# Autodesk Inventor assembly: fourbarintakebearing
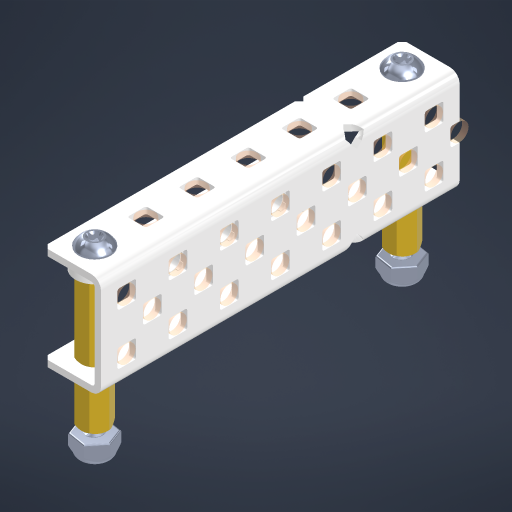
[picture p0: Inventor's stored thumbnail of the model, 512x512]
Saved by Autodesk Inventor 2023 (Build 270158000, 158)
## iProperties
Created: 2023-08-08
Part Number: fourbarintakebearing
Document SubType Name: Assembly
Designer: srbel
Author: srbel
## Documents named in this file (11)
- C:\CAD\OverUnderCAD\Drive\fourbarintakebearing.iam
- C:\CAD\OverUnderCAD\VEX-CAD-Inventor-1.4.0\Structure\C Channel\Aluminum 1x2x1\Alu C 1x2x1x7.ipt
- C:\CAD\OverUnderCAD\VEX-CAD-Inventor-1.4.0\Structure\Standoff\Standoff .50.ipt
- C:\CAD\OverUnderCAD\VEX-CAD-Inventor-1.4.0\Structure\Standoff.ipt
- C:\CAD\OverUnderCAD\VEX-CAD-Inventor-1.4.0\Motion\Spacers\Spacer Nylon .313 OD\NSpacer .313 OD x .125.ipt
- C:\CAD\OverUnderCAD\VEX-CAD-Inventor-1.4.0\Motion\Spacers\Spacer Nylon .313 OD.ipt
- C:\CAD\OverUnderCAD\VEX-CAD-Inventor-1.4.0\Structure\Standoff\Standoff .75.ipt
- C:\CAD\OverUnderCAD\VEX-CAD-Inventor-1.4.0\Motion\Shaft LS\Bearing Flat.ipt
- C:\CAD\OverUnderCAD\VEX-CAD-Inventor-1.4.0\Structure\Hardware\Screw Steel - Star.ipt
- C:\CAD\OverUnderCAD\VEX-CAD-Inventor-1.4.0\Structure\Hardware\Screw Steel - Star\SScrew Star Threaded 1.750.ipt
- C:\CAD\OverUnderCAD\VEX-CAD-Inventor-1.4.0\Structure\Hardware\Nut Thin Nylock.ipt
## Components (12 placed, 7 different names)
1. Alu C 1x2x1x7:1 — Insert:9, Insert:12
2. Standoff .50:1 — Insert:10
3. Standoff .50:2 — Insert:11
4. NSpacer .313 OD x .125:1
5. Standoff .75:3
6. NSpacer .313 OD x .125:2
7. Standoff .75:4
8. Bearing Flat:1
9. SScrew Star Threaded 1.750:2 — Insert:9
10. Nut Thin Nylock:1 — Insert:10
11. Nut Thin Nylock:2 — Insert:11
12. SScrew Star Threaded 1.750:3 — Insert:12
## Relationships (12: Insert 12)
- [Insert]: Alu C 1x2x1x7:1 ↔ Standoff .50:1
- [Insert]: Alu C 1x2x1x7:1 ↔ Standoff .50:2
- [Insert]: NSpacer .313 OD x .125:1 ↔ Standoff .75:3
- [Insert]: Alu C 1x2x1x7:1 ↔ NSpacer .313 OD x .125:1
- [Insert]: NSpacer .313 OD x .125:2 ↔ Standoff .75:4
- [Insert]: Alu C 1x2x1x7:1 ↔ NSpacer .313 OD x .125:2
- [Insert]: Alu C 1x2x1x7:1 ↔ Bearing Flat:1
- [Insert]: Alu C 1x2x1x7:1 ↔ Bearing Flat:1
- Insert:9: Alu C 1x2x1x7:1 ↔ SScrew Star Threaded 1.750:2
- Insert:10 (1.5875 mm): Standoff .50:1 ↔ Nut Thin Nylock:1
- Insert:11 (1.5875 mm): Standoff .50:2 ↔ Nut Thin Nylock:2
- Insert:12: Alu C 1x2x1x7:1 ↔ SScrew Star Threaded 1.750:3
## Named parameters: d294_d1 = 0 mm, d296_d1 = 0 mm
